# Autodesk Inventor assembly: Braço Robô - Assemblagem
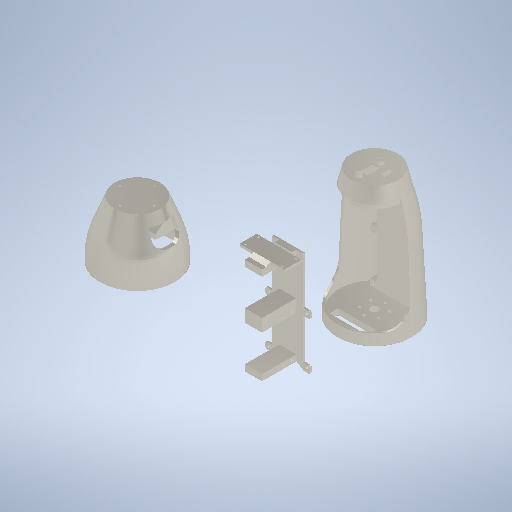
[picture p0: Inventor's stored thumbnail of the model, 512x512]
Saved by Autodesk Inventor 2025.2 (Build 292293000, 293)
## iProperties
Created: 2025-05-20
Part Number: Braço Robô - Assemblagem
Document SubType Name: Assembly
Designer: Formação
Author: Formação
## Documents named in this file (5)
- C:\Users\Formação\Documents\Inventor\Mão_Robô_EMG\Braço Robô - Assemblagem.iam
- C:\Users\Formação\Documents\Inventor\Mão_Robô_EMG\forarm-9-2.ipt
- C:\Users\Formação\Documents\Inventor\Mão_Robô_EMG\forearm9-1.ipt
- C:\Users\Formação\Documents\Inventor\Mão_Robô_EMG\forarm-9-3.ipt
- C:\Users\Formação\Documents\Inventor\Mão_Robô_EMG\servo-hold.ipt
## Components (4 placed, 4 different names)
1. forarm-9-2:1 — Coincidente:1, Coincidente:2, Alinhado:1, Coincidente:3, Alinhado:2, Alinhado:3
2. forearm9-1:1
3. forarm-9-3:1 — Coincidente:3, Alinhado:2, Alinhado:3
4. servo-hold:1
## Relationships (6: Mate 3, Flush 3)
- Coincidente:1 [Mate]: forarm-9-2:1
- Coincidente:2 [Mate]: forarm-9-2:1
- Alinhado:1 [Flush]: forarm-9-2:1
- Coincidente:3 [Mate]: forarm-9-2:1 ↔ forarm-9-3:1
- Alinhado:2 [Flush]: forarm-9-2:1 ↔ forarm-9-3:1
- Alinhado:3 [Flush]: forarm-9-2:1 ↔ forarm-9-3:1
